# Autodesk Inventor assembly: Gel on the limiter
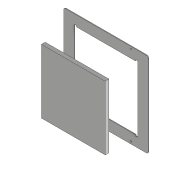
[picture p0: Inventor's stored thumbnail of the model, 180x180]
Saved by Autodesk Inventor 2020 (Build 240168000, 168)
## iProperties
Created: 2022-04-26
Part Number: Gel on the limiter
Document SubType Name: Assembly
Designer: ferrerx
Author: ferrerx
## Documents named in this file (3)
- C:\Users\ferrerx\Desktop\Projects\Boulton Lab\Gel on the limiter.iam
- C:\Users\ferrerx\Desktop\Projects\Boulton Lab\Limiter.ipt
- C:\Users\ferrerx\Desktop\Projects\Boulton Lab\Gel.ipt
## Components (2 placed, 2 different names)
1. Limiter:1 — Mate:1, Mate:2
2. Gel:1 — Mate:1, Mate:2
## Relationships (2: Mate 2)
- Mate:1: Limiter:1 ↔ Gel:1
- Mate:2: Limiter:1 ↔ Gel:1
